# Autodesk Inventor assembly: wheel single
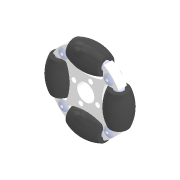
[picture p0: Inventor's stored thumbnail of the model, 180x180]
Saved by Autodesk Inventor 2020 (Build 240168000, 168)
## iProperties
Created: 2019-10-31
Part Number: wheel single
Document SubType Name: Assembly
Designer: ball
Author: ball
Revision Number: ÈÎºÎ
## Documents named in this file (7)
- C:\FTC\FTC8863CAD\2019 Robot\Odoemetry module\wheel single.iam
- C:\FTC\FTC8863CAD\2019 Robot\Odoemetry module\1.5´ç90¶ÈÂÖ¹Ì¶¨°å.ipt
- C:\FTC\FTC8863CAD\2019 Robot\Odoemetry module\1.5´ç90¶ÈÂÖ¹Ì¶¨±ßÆ¬.ipt
- C:\FTC\FTC8863CAD\2019 Robot\Odoemetry module\1.5´ç90¶ÈÂÖÐ¡ÂÖÖá.ipt
- C:\FTC\FTC8863CAD\2019 Robot\Odoemetry module\1.5´ç90¶È»¡ÐÎÂÖ.ipt
- C:\FTC\FTC8863CAD\2019 Robot\Odoemetry module\1.5´ç90¶ÈÂÖÈü¸ÖÌ×.ipt
- C:\FTC\FTC8863CAD\2019 Robot\Odoemetry module\wheel rivet.ipt
## Components (23 placed, 20 different names)
1. 1.5´ç90¶ÈÂÖ¹Ì¶¨°å_16 — Mate:1, Mate:3
2. 1.5´ç90¶ÈÂÖ¹Ì¶¨±ßÆ¬_17 — Mate:2, Mate:4, Mate:5, Mate:6, Mate:7, Mate:8
3. 1.5´ç90¶ÈÂÖ¹Ì¶¨±ßÆ¬_18
4. 1.5´ç90¶ÈÂÖÐ¡ÂÖÖá_19
5. 1.5´ç90¶È»¡ÐÎÂÖ_20
6. 1.5´ç90¶ÈÂÖÈü¸ÖÌ×_21
7. 1.5´ç90¶ÈÂÖÈü¸ÖÌ×_22
8. 1.5´ç90¶ÈÂÖÐ¡ÂÖÖá_23
9. 1.5´ç90¶ÈÂÖÐ¡ÂÖÖá_24
10. 1.5´ç90¶ÈÂÖÐ¡ÂÖÖá_25
11. 1.5´ç90¶ÈÂÖÈü¸ÖÌ×_26
12. 1.5´ç90¶ÈÂÖÈü¸ÖÌ×_27
13. 1.5´ç90¶ÈÂÖÈü¸ÖÌ×_28
14. 1.5´ç90¶ÈÂÖÈü¸ÖÌ×_29
15. 1.5´ç90¶ÈÂÖÈü¸ÖÌ×_30
16. 1.5´ç90¶ÈÂÖÈü¸ÖÌ×_31
17. 1.5´ç90¶È»¡ÐÎÂÖ_32
18. 1.5´ç90¶È»¡ÐÎÂÖ_33
19. 1.5´ç90¶È»¡ÐÎÂÖ_34
20. wheel rivet:1 — Mate:1, Mate:2
21. wheel rivet:2 — Mate:6, Mate:8
22. wheel rivet:3 — Mate:4, Mate:5
23. wheel rivet:4 — Mate:3, Mate:7
## Relationships (8: Mate 8)
- Mate:1: 1.5´ç90¶ÈÂÖ¹Ì¶¨°å_16 ↔ wheel rivet:1
- Mate:2: 1.5´ç90¶ÈÂÖ¹Ì¶¨±ßÆ¬_17 ↔ wheel rivet:1
- Mate:3: 1.5´ç90¶ÈÂÖ¹Ì¶¨°å_16 ↔ wheel rivet:4
- Mate:4: 1.5´ç90¶ÈÂÖ¹Ì¶¨±ßÆ¬_17 ↔ wheel rivet:3
- Mate:5: 1.5´ç90¶ÈÂÖ¹Ì¶¨±ßÆ¬_17 ↔ wheel rivet:3
- Mate:6: 1.5´ç90¶ÈÂÖ¹Ì¶¨±ßÆ¬_17 ↔ wheel rivet:2
- Mate:7: 1.5´ç90¶ÈÂÖ¹Ì¶¨±ßÆ¬_17 ↔ wheel rivet:4
- Mate:8: 1.5´ç90¶ÈÂÖ¹Ì¶¨±ßÆ¬_17 ↔ wheel rivet:2
